# Autodesk Inventor assembly: Butler_assembly
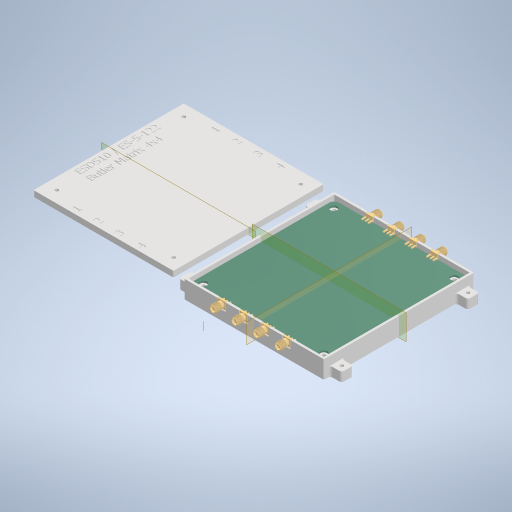
[picture p0: Inventor's stored thumbnail of the model, 512x512]
Saved by Autodesk Inventor 2023.5 (Build 275446000, 446)
## iProperties
Created: 2025-10-09
Part Number: Butler_assembly
Document SubType Name: Assembly
Designer: Mikke
Author: Mikke
## Documents named in this file (4)
- C:\Users\Mikke\OneDrive - Aalborg Universitet\ESD 510 - General\Projekt\Inventor\Butler_matrix\Butler_assembly.iam
- C:\Users\Mikke\OneDrive - Aalborg Universitet\ESD 510 - General\Projekt\Inventor\Butler_matrix\Case.ipt
- C:\Users\Mikke\OneDrive - Aalborg Universitet\ESD 510 - General\Projekt\Inventor\Butler_matrix\Butler_matrix\Butler_matrix.ipt
- C:\Users\Mikke\OneDrive - Aalborg Universitet\ESD 510 - General\Projekt\Inventor\Butler_matrix\Cover_acryl.ipt
## Components (3 placed, 3 different names)
1. Case:1 — Mate:1, Mate:2, Mate:3
2. Butler_matrix:1 — Mate:1, Mate:2, Mate:3, Mate:4
3. Cover_acryl:1 — Mate:4
## Relationships (4: Mate 4)
- Mate:1: Case:1 ↔ Butler_matrix:1
- Mate:2: Case:1 ↔ Butler_matrix:1
- Mate:3: Case:1 ↔ Butler_matrix:1
- Mate:4: Butler_matrix:1 ↔ Cover_acryl:1
